# Autodesk Inventor assembly: XcolumAssy
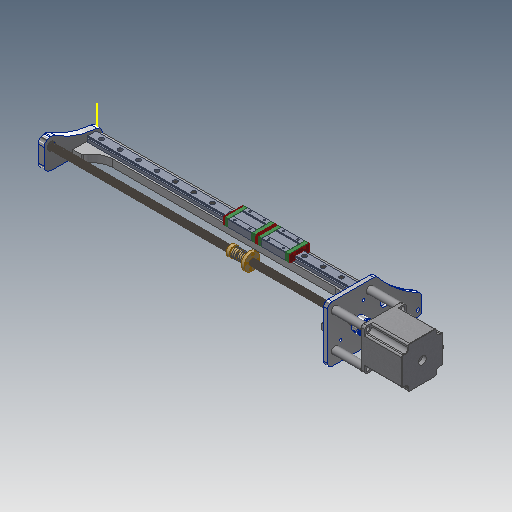
[picture p0: Inventor's stored thumbnail of the model, 512x512]
Saved by Autodesk Inventor 2019 (Build 230136000, 136)
## iProperties
Created: 2018-12-02
Part Number: XcolumAssy
Document SubType Name: Assembly
Designer: LillaHunden
Mass: 1201.08 g
Surface Area: 1709.59 cm^2
Volume: 503.245 cm^3
Density: 2.38666 g/cm^3
Author: LillaHunden
## Documents named in this file (17)
- C:\Users\LillaHunden\Documents\Inventor\3dprinter\3dPrinter\XcolumAssy.iam
- C:\Users\LillaHunden\Documents\Inventor\3dprinter\3dPrinter\Xcolum.ipt
- C:\Users\LillaHunden\Documents\Inventor\3dprinter\3dPrinter\Linear Rials import\Rail X.ipt
- C:\Users\LillaHunden\Documents\Inventor\3dprinter\3dPrinter\XcolBracket.ipt
- C:\Users\LillaHunden\Documents\Inventor\3dprinter\3dPrinter\XMotorMount.ipt
- C:\Users\LillaHunden\Documents\Inventor\3dprinter\3dPrinter\XbearingBracket.ipt
- C:\Users\LillaHunden\Documents\Inventor\3dprinter\3dPrinter\Linear Rials import\MGN block.iam
- C:\Users\LillaHunden\Documents\Inventor\3dprinter\3dPrinter\Linear Rials import\TR8_8(P4) Antibacklash Nut w. spring.ipt
- C:\Users\LillaHunden\Documents\Inventor\3dprinter\3dPrinter\Trapezoidal lead screw tr8x8-4 X.ipt
- C:\Users\LillaHunden\Documents\Inventor\3dprinter\3dPrinter\FR168ZZ flangde bearing.ipt
- C:\Users\LillaHunden\Documents\Inventor\3dprinter\3dPrinter\XMotorStandoff.ipt
- C:\Users\LillaHunden\Documents\Inventor\3dprinter\3dPrinter\23hs6403.ipt
- C:\Users\LillaHunden\Documents\Inventor\Content Center Files\R2019\en-US\DIN 912\DIN 912 - M3 x 0,5 x 10 x 8,75.ipt
- C:\Users\LillaHunden\Documents\Inventor\3dprinter\3dPrinter\coupler.ipt
- C:\Users\LillaHunden\Documents\Inventor\3dprinter\3dPrinter\Nema17 import\Nema 17HS4401-S.ipt
- C:\Users\LillaHunden\Documents\Inventor\3dprinter\3dPrinter\Xfordring.ipt
- C:\Users\LillaHunden\Documents\Inventor\Content Center Files\R2019\en-US\DIN 439-2\DIN 439 - M6 x 1.ipt
## Components (41 placed, 16 different names)
1. Xcolum:1 — Mate:1, Mate:2, Mate:3, Mate:4, Mate:5, Angle:1, Mate:6, Mate:7, Mate:8, Mate:15, Insert:5, Insert:6, Insert:7, Insert:8
2. Rail X:1 — Mate:1, Mate:2, Mate:14, Mate:15, Mate:16, Insert:9, Insert:10, Insert:11, Insert:12, Insert:13, Insert:14, Insert:15, Insert:16, Insert:17, Insert:18, Insert:19, Insert:20
3. XcolBracket:1 — Angle:1, Mate:6, Mate:7, Angle:2
4. XMotorMount:1 — Angle:2, Mate:8, Angle:3, Angle:4, Tangent:1, Angle:5, Tangent:2, Mate:27, Mate:33, Mate:34, Mate:35, Angle:6, Mate:36, Mate:37, Mate:38
5. XbearingBracket:1 — Mate:3, Mate:4, Mate:5, Mate:10, Mate:11, Insert:1, Insert:2, Insert:3, Insert:4
6. MGN block:1 [sub-assembly] — Flush:1, Flush:2, Mate:14, Mate:29
7. MGN block:2 [sub-assembly] — Flush:1, Flush:2, Mate:16, Mate:29, Flush:3
8. TR8_8(P4) Antibacklash Nut w. spring:1 — Cylindrical:1, Flush:3
9. Trapezoidal lead screw tr8x8-4 X:1 — Mate:12, Mate:13, Mate:30, Cylindrical:1, Mate:39
10. FR168ZZ flangde bearing:1 — Mate:10, Mate:11, Mate:12, Mate:13
11. 23hs6403:1 — Angle:3, Mate:30, Mate:31, Mate:32, Mate:38, Mate:40, Mate:41, Mate:42, Mate:43, Mate:44, Mate:45, Mate:46, Mate:47
12. DIN 912 - replaced by DIN EN ISO 4762 M3 x 10:1 — Insert:1
13. DIN 912 - replaced by DIN EN ISO 4762 M3 x 10:2 — Insert:2
14. DIN 912 - replaced by DIN EN ISO 4762 M3 x 10:3 — Insert:3
15. DIN 912 - replaced by DIN EN ISO 4762 M3 x 10:4 — Insert:4
16. DIN 912 - replaced by DIN EN ISO 4762 M3 x 10:5 — Insert:5
17. DIN 912 - replaced by DIN EN ISO 4762 M3 x 10:6 — Insert:6
18. DIN 912 - replaced by DIN EN ISO 4762 M3 x 10:7 — Insert:7
19. DIN 912 - replaced by DIN EN ISO 4762 M3 x 10:8 — Insert:8
20. DIN 912 - replaced by DIN EN ISO 4762 M3 x 10:9 — Insert:9
21. DIN 912 - replaced by DIN EN ISO 4762 M3 x 10:10 — Insert:10
22. DIN 912 - replaced by DIN EN ISO 4762 M3 x 10:11 — Insert:11
23. DIN 912 - replaced by DIN EN ISO 4762 M3 x 10:12 — Insert:12
24. DIN 912 - replaced by DIN EN ISO 4762 M3 x 10:13 — Insert:13
25. DIN 912 - replaced by DIN EN ISO 4762 M3 x 10:14 — Insert:14
26. DIN 912 - replaced by DIN EN ISO 4762 M3 x 10:15 — Insert:15
27. DIN 912 - replaced by DIN EN ISO 4762 M3 x 10:16 — Insert:16
28. DIN 912 - replaced by DIN EN ISO 4762 M3 x 10:17 — Insert:17
29. DIN 912 - replaced by DIN EN ISO 4762 M3 x 10:18 — Insert:18
30. DIN 912 - replaced by DIN EN ISO 4762 M3 x 10:19 — Insert:19
31. DIN 912 - replaced by DIN EN ISO 4762 M3 x 10:20 — Insert:20
32. FR168ZZ flangde bearing:2 — Mate:27, Mate:31
33. coupler:1 — Mate:32, Mate:33
34. Nema 17HS4401-S:1 — Mate:34, Mate:35, Angle:6
35. FR168ZZ flangde bearing:3 — Mate:36, Mate:37, Insert:21
36. Xfordring:1 — Insert:21
37. DIN 439-2 - replaced by DIN EN 24035/28675 M6:1 — Mate:39
38. XMotorStandoff:1 — Mate:44, Mate:45
39. XMotorStandoff:2 — Mate:40, Mate:41
40. XMotorStandoff:3 — Mate:42, Mate:47
41. XMotorStandoff:4 — Mate:43, Mate:46
## Relationships (69: Mate 35, Insert 21, Angle 6, Flush 3, Tangent 2, Symmetry 1, CylindricalJoint 1)
- Mate:1: Xcolum:1 ↔ Rail X:1
- Mate:2: Xcolum:1 ↔ Rail X:1
- Mate:3: Xcolum:1 ↔ XbearingBracket:1
- Mate:4: Xcolum:1 ↔ XbearingBracket:1
- Mate:5: Xcolum:1 ↔ XbearingBracket:1
- Angle:1 (0 deg): Xcolum:1 ↔ XcolBracket:1
- Mate:6: Xcolum:1 ↔ XcolBracket:1
- Mate:7: Xcolum:1 ↔ XcolBracket:1
- Angle:2 (0 deg): XcolBracket:1 ↔ XMotorMount:1
- Mate:8: Xcolum:1 ↔ XMotorMount:1
- Mate:10: XbearingBracket:1 ↔ FR168ZZ flangde bearing:1
- Mate:11: XbearingBracket:1 ↔ FR168ZZ flangde bearing:1
- Mate:12: Trapezoidal lead screw tr8x8-4 X:1 ↔ FR168ZZ flangde bearing:1
- Mate:13: Trapezoidal lead screw tr8x8-4 X:1 ↔ FR168ZZ flangde bearing:1
- Flush:1: MGN block:1 ↔ MGN block:2
- Flush:2: MGN block:1 ↔ MGN block:2
- Mate:14: Rail X:1 ↔ MGN block:1
- Mate:15: Xcolum:1 ↔ Rail X:1
- Mate:16: Rail X:1 ↔ MGN block:2
- Insert:1: XbearingBracket:1 ↔ DIN 912 - replaced by DIN EN ISO 4762 M3 x 10:1
- Insert:2: XbearingBracket:1 ↔ DIN 912 - replaced by DIN EN ISO 4762 M3 x 10:2
- Insert:3: XbearingBracket:1 ↔ DIN 912 - replaced by DIN EN ISO 4762 M3 x 10:3
- Insert:4: XbearingBracket:1 ↔ DIN 912 - replaced by DIN EN ISO 4762 M3 x 10:4
- Insert:5: Xcolum:1 ↔ DIN 912 - replaced by DIN EN ISO 4762 M3 x 10:5
- Insert:6: Xcolum:1 ↔ DIN 912 - replaced by DIN EN ISO 4762 M3 x 10:6
- Insert:7: Xcolum:1 ↔ DIN 912 - replaced by DIN EN ISO 4762 M3 x 10:7
- Insert:8: Xcolum:1 ↔ DIN 912 - replaced by DIN EN ISO 4762 M3 x 10:8
- Insert:9: Rail X:1 ↔ DIN 912 - replaced by DIN EN ISO 4762 M3 x 10:9
- Insert:10: Rail X:1 ↔ DIN 912 - replaced by DIN EN ISO 4762 M3 x 10:10
- Insert:11: Rail X:1 ↔ DIN 912 - replaced by DIN EN ISO 4762 M3 x 10:11
- Insert:12: Rail X:1 ↔ DIN 912 - replaced by DIN EN ISO 4762 M3 x 10:12
- Insert:13: Rail X:1 ↔ DIN 912 - replaced by DIN EN ISO 4762 M3 x 10:13
- Insert:14: Rail X:1 ↔ DIN 912 - replaced by DIN EN ISO 4762 M3 x 10:14
- Insert:15: Rail X:1 ↔ DIN 912 - replaced by DIN EN ISO 4762 M3 x 10:15
- Insert:16: Rail X:1 ↔ DIN 912 - replaced by DIN EN ISO 4762 M3 x 10:16
- Insert:17: Rail X:1 ↔ DIN 912 - replaced by DIN EN ISO 4762 M3 x 10:17
- Insert:18: Rail X:1 ↔ DIN 912 - replaced by DIN EN ISO 4762 M3 x 10:18
- Insert:19: Rail X:1 ↔ DIN 912 - replaced by DIN EN ISO 4762 M3 x 10:19
- Insert:20: Rail X:1 ↔ DIN 912 - replaced by DIN EN ISO 4762 M3 x 10:20
- Angle:3 (270 deg): XMotorMount:1 ↔ 23hs6403:1
- Angle:4 (0 deg): XMotorMount:1
- Tangent:1: XMotorMount:1
- Angle:5 (0 deg): XMotorMount:1
- Tangent:2: XMotorMount:1
- Symmetry:1
- Mate:27: XMotorMount:1 ↔ FR168ZZ flangde bearing:2
- Mate:29 (1.5 mm): MGN block:1 ↔ MGN block:2
- Mate:30: Trapezoidal lead screw tr8x8-4 X:1 ↔ 23hs6403:1
- Mate:31: 23hs6403:1 ↔ FR168ZZ flangde bearing:2
- Mate:32: 23hs6403:1 ↔ coupler:1
- Mate:33 (8 mm): XMotorMount:1 ↔ coupler:1
- Mate:34: XMotorMount:1 ↔ Nema 17HS4401-S:1
- Mate:35: XMotorMount:1 ↔ Nema 17HS4401-S:1
- Angle:6 (0 deg): XMotorMount:1 ↔ Nema 17HS4401-S:1
- Cylindrical:1: TR8_8(P4) Antibacklash Nut w. spring:1 ↔ Trapezoidal lead screw tr8x8-4 X:1
- Mate:36: XMotorMount:1 ↔ FR168ZZ flangde bearing:3
- Mate:37: XMotorMount:1 ↔ FR168ZZ flangde bearing:3
- Mate:38 (40 mm): XMotorMount:1 ↔ 23hs6403:1
- Mate:39: Trapezoidal lead screw tr8x8-4 X:1 ↔ DIN 439-2 - replaced by DIN EN 24035/28675 M6:1
- Insert:21: FR168ZZ flangde bearing:3 ↔ Xfordring:1
- Mate:40: 23hs6403:1 ↔ XMotorStandoff:2
- Mate:41: 23hs6403:1 ↔ XMotorStandoff:2
- Mate:42: 23hs6403:1 ↔ XMotorStandoff:3
- Mate:43: 23hs6403:1 ↔ XMotorStandoff:4
- Mate:44: 23hs6403:1 ↔ XMotorStandoff:1
- Mate:45: 23hs6403:1 ↔ XMotorStandoff:1
- Mate:46: 23hs6403:1 ↔ XMotorStandoff:4
- Mate:47: 23hs6403:1 ↔ XMotorStandoff:3
- Flush:3 (11 mm): MGN block:2 ↔ TR8_8(P4) Antibacklash Nut w. spring:1
